# Autodesk Inventor assembly: Galileo Chain Anchor China
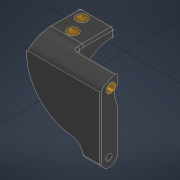
[picture p0: Inventor's stored thumbnail of the model, 180x180]
Saved by Autodesk Inventor 2022.2 (Build 262287010, 287A)
## iProperties
Created: 2022-03-15
Part Number: Galileo Chain Anchor China
Document SubType Name: Assembly
Designer: sleib
Author: sleib
## Documents named in this file (3)
- C:\Users\sleib\Projekte\Voron-2\CAD\Inventor\Galileo Clockwork\Galileo Chain Anchor China.iam
- C:\Users\sleib\Projekte\Voron-2\CAD\Inventor\Galileo Clockwork\China Anchor.ipt
- C:\Users\sleib\Projekte\Voron-2\CAD\Inventor\M3 Threaded Insert.ipt
## Components (4 placed, 2 different names)
1. China Anchor:1 — Passend:1, Passend:2, Passend:3, Fluchtend:1, Fluchtend:2, Fluchtend:3
2. M3 Threaded Insert:1 — Passend:2, Fluchtend:2
3. M3 Threaded Insert:2 — Passend:3, Fluchtend:1
4. M3 Threaded Insert:3 — Passend:1, Fluchtend:3
## Relationships (6: Mate 3, Flush 3)
- Passend:1 [Mate]: China Anchor:1 ↔ M3 Threaded Insert:3
- Passend:2 [Mate]: China Anchor:1 ↔ M3 Threaded Insert:1
- Passend:3 [Mate]: China Anchor:1 ↔ M3 Threaded Insert:2
- Fluchtend:1 [Flush]: China Anchor:1 ↔ M3 Threaded Insert:2
- Fluchtend:2 [Flush]: China Anchor:1 ↔ M3 Threaded Insert:1
- Fluchtend:3 [Flush]: China Anchor:1 ↔ M3 Threaded Insert:3
